# Autodesk Inventor assembly: +XPanel
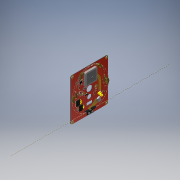
[picture p0: Inventor's stored thumbnail of the model, 180x180]
Saved by Autodesk Inventor 2018 (Build 220112000, 112)
## iProperties
Created: 2018-10-25
Part Number: +XPanel
Document SubType Name: Assembly
Designer: Bradley
Author: Bradley
## Documents named in this file (28)
- C:\Users\Bradley\Documents\GitHub\CougSat1-Hardware\CougSat1-RadioBoard\CADModel\Native\+XPanel.iam
- C:\Users\Bradley\Documents\GitHub\CougSat1-Hardware\CougSat1-RadioBoard\CADModel\Native\+XPanel_PCB.ipt
- C:\Users\Bradley\Documents\GitHub\CougSat1-Hardware\CougSat1-RadioBoard\CADModel\Native\+XPanel_AntennaPost.ipt
- C:\Users\Bradley\Documents\GitHub\CougSat1-Hardware\CougSat1-RadioBoard\CADModel\Native\+XPanel_AntennaMount.ipt
- C:\Users\Bradley\Documents\GitHub\CougSat1-Hardware\CougSat1-RadioBoard\CADModel\Native\+XPanel_AntennaStored+Y.ipt
- C:\Users\Bradley\Documents\GitHub\CougSat1-Hardware\CougSat1-RadioBoard\CADModel\Native\+XPanel_AntennaStored-Y.ipt
- C:\Users\Bradley\Documents\GitHub\CougSat1-Hardware\CougSat1-RadioBoard\CADModel\Native\+XPanel_AntennaDeployed.ipt
- C:\Users\Bradley\Documents\GitHub\Resources\SupplierDocuments\04 - Connectors SMT\04-0001\04-0001.iam
- C:\Users\Bradley\Documents\GitHub\Resources\SupplierDocuments\04 - Connectors SMT\04-0008\04-0008.iam
- C:\Users\Bradley\Documents\GitHub\Resources\SupplierDocuments\65 - RF\65-0010\65-0010.ipt
- C:\Users\Bradley\Documents\GitHub\Resources\SupplierDocuments\48 - Hardware\48-0240\48-0240.ipt
- C:\Users\Bradley\Documents\GitHub\Resources\SupplierDocuments\48 - Hardware\48-0074\48-0074.ipt
- C:\Users\Bradley\Documents\GitHub\Resources\SupplierDocuments\21 - Resistor 1608\21-0000\21-0000.ipt
- C:\Users\Bradley\Documents\GitHub\Resources\SupplierDocuments\36 - Ferrite\36-152A\36-152A.ipt
- C:\Users\Bradley\Documents\GitHub\Resources\SupplierDocuments\11 - Capacitor Ceramic 1608\11-105A\11-105A.ipt
- C:\Users\Bradley\Documents\GitHub\Resources\SupplierDocuments\21 - Resistor 1608\21-1001\21-1001.ipt
- C:\Users\Bradley\Documents\GitHub\Resources\SupplierDocuments\21 - Resistor 1608\21-2001\21-2001.ipt
- C:\Users\Bradley\Documents\GitHub\Resources\SupplierDocuments\16 - Capacitor Tantalum SMT\16-475A\16-475A.ipt
- C:\Users\Bradley\Documents\GitHub\Resources\SupplierDocuments\11 - Capacitor Ceramic 1608\11-106A\11-106A.ipt
- C:\Users\Bradley\Documents\GitHub\Resources\SupplierDocuments\21 - Resistor 1608\21-1002\21-1002.ipt
- C:\Users\Bradley\Documents\GitHub\Resources\SupplierDocuments\26 - Resistor Misc\26-0008\26-0008.ipt
- C:\Users\Bradley\Documents\GitHub\Resources\SupplierDocuments\26 - Resistor Misc\26-0001\26-0001.ipt
- C:\Users\Bradley\Documents\GitHub\Resources\SupplierDocuments\11 - Capacitor Ceramic 1608\11-104A\11-104A.ipt
- C:\Users\Bradley\Documents\GitHub\Resources\SupplierDocuments\27 - Conversion IC\27-0003\27-0003.ipt
- C:\Users\Bradley\Documents\GitHub\Resources\SupplierDocuments\08 - Amplifier (excluding RF)\08-0002\08-0002.ipt
- C:\Users\Bradley\Documents\GitHub\Resources\SupplierDocuments\39 - Coils Misc\39-0001\39-0001.ipt
- C:\Users\Bradley\Documents\GitHub\Resources\SupplierDocuments\66 - Sensor\66-0003\66-0003.ipt
- C:\Users\Bradley\Documents\GitHub\Resources\SupplierDocuments\25 - Resistor THT\25-5.00\25-5.00.ipt
## Components (62 placed, 27 different names)
1. 25-5.00:2 — Mate:136, Mate:146, Mate:147, Angle:16
2. 25-5.00:1 — Mate:135, Mate:144, Mate:145, Angle:15
3. 66-0003:1 — Mate:132, Mate:133, Mate:134
4. 48-0074:1 — Insert:9
5. 48-0074:2 — Insert:10
6. 04-0008:1 [sub-assembly] — Mate:130, Flush:36, Flush:37
7. 04-0008:2 [sub-assembly] — Mate:129, Mate:131, Flush:38
8. 65-0010:1 — Mate:128, Flush:34, Flush:35
9. 39-0001:1 — Mate:125, Mate:126, Mate:127, Angle:14
10. 04-0001:1 [sub-assembly] — Mate:5, Flush:3, Mate:6
11. 04-0001:2 [sub-assembly] — Mate:28, Mate:29, Flush:7
12. 27-0003:1 — Mate:122, Mate:124, Flush:31
13. 08-0002:1 — Mate:123, Flush:32, Flush:33
14. 11-104A:1 — Mate:98, Mate:108, Mate:109
15. 11-104A:2 — Mate:99, Mate:110, Flush:25
16. 11-104A:3 — Mate:100, Mate:111, Mate:112
17. 11-104A:4 — Mate:101, Mate:113, Flush:26
18. 11-104A:5 — Mate:102, Mate:114, Mate:115
19. 11-104A:6 — Mate:103, Mate:116, Flush:27
20. 11-104A:7 — Mate:104, Mate:117, Flush:28
21. 11-104A:8 — Mate:105, Mate:118, Mate:119
22. 11-104A:9 — Mate:106, Mate:120, Flush:29
23. 11-104A:10 — Mate:107, Mate:121, Flush:30
24. 21-0000:1 — Mate:30, Mate:41, Mate:42
25. 21-0000:2 — Mate:31, Mate:43, Flush:8
26. 21-0000:3 — Mate:32, Mate:44, Flush:9
27. 21-0000:4 — Mate:33, Mate:45, Mate:46
28. 21-0000:5 — Mate:34, Mate:47, Flush:10
29. 21-0000:6 — Mate:35, Mate:48, Mate:49
30. 21-0000:7 — Mate:36, Mate:50, Mate:51
31. 21-0000:8 — Mate:37, Mate:52, Flush:11
32. 21-0000:9 — Mate:38, Mate:53, Flush:12
33. 21-0000:10 — Mate:39, Mate:54, Mate:55
34. 21-0000:11 — Mate:40, Mate:56, Flush:13
35. 36-152A:1 — Mate:57, Mate:58, Mate:59
36. 11-105A:1 — Mate:60, Mate:61, Mate:62
37. 21-1001:1 — Mate:63, Mate:65, Flush:14
38. 21-2001:1 — Mate:64, Mate:66, Flush:15
39. 16-475A:1 — Mate:67, Flush:16, Flush:17
40. 11-106A:1 — Mate:68, Mate:69, Flush:18
41. 21-1002:1 — Mate:70, Mate:148, Flush:44
42. 21-1002:2 — Mate:71, Mate:74, Mate:75
43. 26-0008:1 — Mate:76, Mate:83, Mate:84
44. 26-0008:2 — Mate:77, Mate:85, Flush:19
45. 26-0008:3 — Mate:78, Mate:86, Flush:20
46. 26-0008:4 — Mate:79, Mate:87, Flush:21
47. 26-0008:5 — Mate:80, Mate:88, Flush:22
48. 26-0008:6 — Mate:81, Mate:89, Flush:23
49. 26-0008:7 — Mate:82, Mate:90, Flush:24
50. 26-0001:1 — Mate:91, Mate:92, Mate:93
51. 48-0240:1 — Insert:13
52. 48-0240:2 — Insert:14
53. +XPanel_AntennaDeployed:1 — Mate:25, Mate:141
54. +XPanel_AntennaDeployed:2 — Mate:27, Mate:142
55. +XPanel_AntennaMount:1 — Insert:11, Insert:12, Insert:13, Insert:14, Mate:25, Mate:27
56. +XPanel_AntennaPost:1 — Insert:4, Angle:10
57. +XPanel_AntennaPost:2 — Insert:8, Angle:11
58. +XPanel_AntennaPost:3 — Insert:7, Angle:12
59. +XPanel_AntennaPost:4 — Insert:6, Angle:13
60. +XPanel_AntennaStored+Y:1 — Flush:39, Flush:40, Flush:41, Flush:43
61. +XPanel_AntennaStored-Y:1 — Mate:143, Flush:42, Flush:43
62. +XPanel_PCB:1 — Insert:4, Insert:6, Insert:7, Insert:8, Insert:9, Insert:10, Insert:11, Mate:5, Mate:28, Mate:30, Mate:31, Mate:32, Mate:33, Mate:34, Mate:35, Mate:36, Mate:37, Mate:38, Mate:39, Mate:40, Mate:57, Mate:60, Mate:63, Mate:64, Mate:67, Mate:68, Mate:70, Mate:71, Mate:76, Mate:77, Mate:78, Mate:79, Mate:80, Mate:81, Mate:82, Mate:91, Mate:98, Mate:99, Mate:100, Mate:101, Mate:102, Mate:103, Mate:104, Mate:105, Mate:106, Mate:107, Mate:122, Mate:123, Mate:125, Mate:128, Mate:129, Mate:130, Mate:132, Mate:135, Mate:136, Mate:141, Mate:142, Flush:41, Insert:12
## Relationships (171: Mate 115, Flush 39, Insert 10, Angle 7)
- Insert:4: +XPanel_AntennaPost:1 ↔ +XPanel_PCB:1
- Insert:6: +XPanel_AntennaPost:4 ↔ +XPanel_PCB:1
- Insert:7: +XPanel_AntennaPost:3 ↔ +XPanel_PCB:1
- Insert:8: +XPanel_AntennaPost:2 ↔ +XPanel_PCB:1
- Insert:9: 48-0074:1 ↔ +XPanel_PCB:1
- Insert:10: 48-0074:2 ↔ +XPanel_PCB:1
- Insert:11: +XPanel_AntennaMount:1 ↔ +XPanel_PCB:1
- Insert:12: +XPanel_AntennaMount:1 ↔ +XPanel_PCB:1
- Insert:13: 48-0240:1 ↔ +XPanel_AntennaMount:1
- Insert:14: 48-0240:2 ↔ +XPanel_AntennaMount:1
- Mate:5: 04-0001:1 ↔ +XPanel_PCB:1
- Flush:3 (23 mm): 04-0001:1
- Mate:6 (-23 mm): 04-0001:1
- Angle:10 (90 deg): +XPanel_AntennaPost:1
- Angle:11 (-90 deg): +XPanel_AntennaPost:2
- Angle:12 (45 deg): +XPanel_AntennaPost:3
- Angle:13 (-45 deg): +XPanel_AntennaPost:4
- Mate:25: +XPanel_AntennaDeployed:1 ↔ +XPanel_AntennaMount:1
- Mate:27: +XPanel_AntennaDeployed:2 ↔ +XPanel_AntennaMount:1
- Mate:28: 04-0001:2 ↔ +XPanel_PCB:1
- Mate:29 (-11 mm): 04-0001:2
- Flush:7 (29 mm): 04-0001:2
- Mate:30: 21-0000:1 ↔ +XPanel_PCB:1
- Mate:31: 21-0000:2 ↔ +XPanel_PCB:1
- Mate:32: 21-0000:3 ↔ +XPanel_PCB:1
- Mate:33: 21-0000:4 ↔ +XPanel_PCB:1
- Mate:34: 21-0000:5 ↔ +XPanel_PCB:1
- Mate:35: 21-0000:6 ↔ +XPanel_PCB:1
- Mate:36: 21-0000:7 ↔ +XPanel_PCB:1
- Mate:37: 21-0000:8 ↔ +XPanel_PCB:1
- Mate:38: 21-0000:9 ↔ +XPanel_PCB:1
- Mate:39: 21-0000:10 ↔ +XPanel_PCB:1
- Mate:40: 21-0000:11 ↔ +XPanel_PCB:1
- Mate:41 (-16.4 mm): 21-0000:1
- Mate:42 (5.2 mm): 21-0000:1
- Mate:43 (22 mm): 21-0000:2
- Flush:8 (23.5 mm): 21-0000:2
- Mate:44 (22 mm): 21-0000:3
- Flush:9 (25.25 mm): 21-0000:3
- Mate:45 (28.6 mm): 21-0000:4
- Mate:46 (-18 mm): 21-0000:4
- Mate:47 (-5.25 mm): 21-0000:5
- Flush:10 (-13 mm): 21-0000:5
- Mate:48 (-19.1 mm): 21-0000:6
- Mate:49 (-1 mm): 21-0000:6
- Mate:50 (-27.5 mm): 21-0000:7
- Mate:51 (-20.8 mm): 21-0000:7
- Mate:52 (25 mm): 21-0000:8
- Flush:11 (23.5 mm): 21-0000:8
- Mate:53 (26.5 mm): 21-0000:9
- Flush:12 (27 mm): 21-0000:9
- Mate:54 (32.8 mm): 21-0000:10
- Mate:55 (-18.9 mm): 21-0000:10
- Mate:56 (25 mm): 21-0000:11
- Flush:13 (25.25 mm): 21-0000:11
- Mate:57: 36-152A:1 ↔ +XPanel_PCB:1
- Mate:58 (2.6 mm): 36-152A:1
- Mate:59 (-22.9 mm): 36-152A:1
- Mate:60: 11-105A:1 ↔ +XPanel_PCB:1
- Mate:61 (27.25 mm): 11-105A:1
- Mate:62 (-17.75 mm): 11-105A:1
- Mate:63: 21-1001:1 ↔ +XPanel_PCB:1
- Mate:64: 21-2001:1 ↔ +XPanel_PCB:1
- Mate:65 (18.9 mm): 21-1001:1
- Flush:14 (15.2 mm): 21-1001:1
- Mate:66 (9.4 mm): 21-2001:1
- Flush:15 (4.2 mm): 21-2001:1
- Mate:67: 16-475A:1 ↔ +XPanel_PCB:1
- Flush:16 (20.7 mm): 16-475A:1
- Flush:17 (-6.1 mm): 16-475A:1
- Mate:68: 11-106A:1 ↔ +XPanel_PCB:1
- Mate:69 (-15.25 mm): 11-106A:1
- Flush:18 (-26.75 mm): 11-106A:1
- Mate:70: 21-1002:1 ↔ +XPanel_PCB:1
- Mate:71: 21-1002:2 ↔ +XPanel_PCB:1
- Mate:74 (-25.8 mm): 21-1002:2
- Mate:75 (-22.7 mm): 21-1002:2
- Mate:76: 26-0008:1 ↔ +XPanel_PCB:1
- Mate:77: 26-0008:2 ↔ +XPanel_PCB:1
- Mate:78: 26-0008:3 ↔ +XPanel_PCB:1
- Mate:79: 26-0008:4 ↔ +XPanel_PCB:1
- Mate:80: 26-0008:5 ↔ +XPanel_PCB:1
- Mate:81: 26-0008:6 ↔ +XPanel_PCB:1
- Mate:82: 26-0008:7 ↔ +XPanel_PCB:1
- Mate:83 (3.5 mm): 26-0008:1
- Mate:84 (-26.2 mm): 26-0008:1
- Mate:85 (9.75 mm): 26-0008:2
- Flush:19 (9 mm): 26-0008:2
- Mate:86 (10 mm): 26-0008:3
- Flush:20 (14 mm): 26-0008:3
- Mate:87 (10 mm): 26-0008:4
- Flush:21 (12.25 mm): 26-0008:4
- Mate:88 (-22 mm): 26-0008:5
- Flush:22 (-29 mm): 26-0008:5
- Mate:89 (13.25 mm): 26-0008:6
- Flush:23 (9 mm): 26-0008:6
- Mate:90 (-14.5 mm): 26-0008:7
- Flush:24 (-23.25 mm): 26-0008:7
- Mate:91: 26-0001:1 ↔ +XPanel_PCB:1
- Mate:92 (-7.3 mm): 26-0001:1
- Mate:93 (-5 mm): 26-0001:1
- Mate:98: 11-104A:1 ↔ +XPanel_PCB:1
- Mate:99: 11-104A:2 ↔ +XPanel_PCB:1
- Mate:100: 11-104A:3 ↔ +XPanel_PCB:1
- Mate:101: 11-104A:4 ↔ +XPanel_PCB:1
- Mate:102: 11-104A:5 ↔ +XPanel_PCB:1
- Mate:103: 11-104A:6 ↔ +XPanel_PCB:1
- Mate:104: 11-104A:7 ↔ +XPanel_PCB:1
- Mate:105: 11-104A:8 ↔ +XPanel_PCB:1
- Mate:106: 11-104A:9 ↔ +XPanel_PCB:1
- Mate:107: 11-104A:10 ↔ +XPanel_PCB:1
- Mate:108 (-5.25 mm): 11-104A:1
- Mate:109 (14.75 mm): 11-104A:1
- Mate:110 (-19.1 mm): 11-104A:2
- Flush:25 (-0.8 mm): 11-104A:2
- Mate:111 (18.9 mm): 11-104A:3
- Mate:112 (-16.9 mm): 11-104A:3
- Mate:113 (-21.7 mm): 11-104A:4
- Flush:26 (-11.5 mm): 11-104A:4
- Mate:114 (27.25 mm): 11-104A:5
- Mate:115 (-19.5 mm): 11-104A:5
- Mate:116 (-20.5 mm): 11-104A:6
- Flush:27 (-3.2 mm): 11-104A:6
- Mate:117 (-27.5 mm): 11-104A:7
- Flush:28 (18.7 mm): 11-104A:7
- Mate:118 (26.5 mm): 11-104A:8
- Mate:119 (-28.7 mm): 11-104A:8
- Mate:120 (33 mm): 11-104A:9
- Flush:29 (9.3 mm): 11-104A:9
- Mate:121 (28.6 mm): 11-104A:10
- Flush:30 (16.2 mm): 11-104A:10
- Mate:122: 27-0003:1 ↔ +XPanel_PCB:1
- Mate:123: 08-0002:1 ↔ +XPanel_PCB:1
- Mate:124 (-18.7 mm): 27-0003:1
- Flush:31 (-23.1 mm): 27-0003:1
- Flush:32 (-15.6 mm): 08-0002:1
- Flush:33 (22.3 mm): 08-0002:1
- Mate:125: 39-0001:1 ↔ +XPanel_PCB:1
- Mate:126 (18.664 mm): 39-0001:1
- Mate:127 (-25.686 mm): 39-0001:1
- Angle:14 (-202 deg): 39-0001:1
- Mate:128: 65-0010:1 ↔ +XPanel_PCB:1
- Flush:34: 65-0010:1
- Flush:35 (-26 mm): 65-0010:1
- Mate:129: 04-0008:2 ↔ +XPanel_PCB:1
- Mate:130: 04-0008:1 ↔ +XPanel_PCB:1
- Flush:36 (14 mm): 04-0008:1
- Flush:37 (-22 mm): 04-0008:1
- Mate:131 (25.5 mm): 04-0008:2
- Flush:38 (22 mm): 04-0008:2
- Mate:132: 66-0003:1 ↔ +XPanel_PCB:1
- Mate:133 (-10.4 mm): 66-0003:1
- Mate:134 (8.6 mm): 66-0003:1
- Mate:135 (2 mm): 25-5.00:1 ↔ +XPanel_PCB:1
- Mate:136 (2 mm): 25-5.00:2 ↔ +XPanel_PCB:1
- Flush:39: +XPanel_AntennaStored+Y:1
- Flush:40: +XPanel_AntennaStored+Y:1
- Mate:141: +XPanel_AntennaDeployed:1 ↔ +XPanel_PCB:1
- Mate:142: +XPanel_AntennaDeployed:2 ↔ +XPanel_PCB:1
- Flush:41 (1 mm): +XPanel_AntennaStored+Y:1 ↔ +XPanel_PCB:1
- Mate:143: +XPanel_AntennaStored-Y:1
- Flush:42: +XPanel_AntennaStored-Y:1
- Flush:43: +XPanel_AntennaStored+Y:1 ↔ +XPanel_AntennaStored-Y:1
- Mate:144 (30 mm): 25-5.00:1
- Mate:145 (6 mm): 25-5.00:1
- Angle:15 (7 deg): 25-5.00:1
- Mate:146 (-30 mm): 25-5.00:2
- Mate:147 (6 mm): 25-5.00:2
- Angle:16 (-7 deg): 25-5.00:2
- Mate:148 (-25.2 mm): 21-1002:1
- Flush:44 (25.6 mm): 21-1002:1
